# Autodesk Inventor assembly: Assembly_USBholder
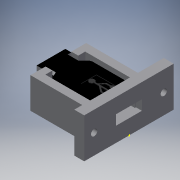
[picture p0: Inventor's stored thumbnail of the model, 180x180]
Saved by Autodesk Inventor 2018 (Build 220112000, 112)
## iProperties
Created: 2018-07-16
Part Number: Assembly_USBholder
Document SubType Name: Assembly
Designer: David
Author: David
## Documents named in this file (3)
- C:\Users\David\Documents\optoelectronics\CAD\usb-better-1.snapshot.4\Assembly_USBholder.iam
- C:\Users\David\Documents\optoelectronics\CAD\usb-better-1.snapshot.4\USB_housing.ipt
- C:\Users\David\Documents\optoelectronics\CAD\usb-better-1.snapshot.4\usb head_V2.ipt
## Components (2 placed, 2 different names)
1. USB_housing:1 — Mate:1, Mate:2
2. usb head_V2:1 — Mate:1, Mate:2
## Relationships (2: Mate 2)
- Mate:1: USB_housing:1 ↔ usb head_V2:1
- Mate:2: USB_housing:1 ↔ usb head_V2:1
